# Autodesk Inventor assembly: tower
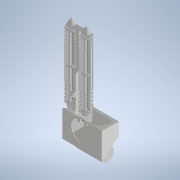
[picture p0: Inventor's stored thumbnail of the model, 180x180]
Saved by Autodesk Inventor 2020.1 (Build 241239000, 239)
## iProperties
Created: 2022-03-20
Part Number: tower
Document SubType Name: Assembly
Designer: User
Author: User
## Documents named in this file (4)
- D:\GitHub\TANK\3D-turret\tower.iam
- D:\GitHub\TANK\3D-turret\full guns.iam
- D:\GitHub\TANK\3D-turret\кольцо башни.ipt
- D:\GitHub\TANK\3D-turret\ось крепление пушки.ipt
## Components (3 placed, 3 different names)
1. full guns:1 [sub-assembly] — С поворотом:1
2. кольцо башни:1 — Жесткий:1, С поворотом:1
3. ось крепление пушки:1 — Жесткий:1
## Relationships (2: WeldJoint 1, RevoluteJoint 1)
- Жесткий:1 [WeldJoint]: кольцо башни:1 ↔ ось крепление пушки:1
- С поворотом:1 [RevoluteJoint]: full guns:1 ↔ кольцо башни:1
